# Autodesk Inventor assembly: iceTubeClockAssembly
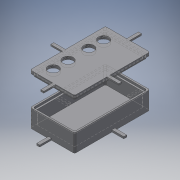
[picture p0: Inventor's stored thumbnail of the model, 180x180]
Saved by Autodesk Inventor 2016 (Build 200138000, 138)
## iProperties
Created: 2016-04-01
Part Number: iceTubeClockAssembly
Document SubType Name: Assembly
Designer: boztalay
Author: boztalay
## Documents named in this file (3)
- \\engin-labs.m.storage.umich.edu\boztalay\iceTubeClockAssembly.iam
- \\engin-labs.m.storage.umich.edu\boztalay\iceTubeClockBase.ipt
- \\engin-labs.m.storage.umich.edu\boztalay\iceTubeClockTop.ipt
## Components (2 placed, 2 different names)
1. iceTubeClockBase:1 — Mate:1, Flush:1, Flush:2
2. iceTubeClockTop:1 — Mate:1, Flush:1, Flush:2
## Relationships (3: Flush 2, Mate 1)
- Mate:1 (63.5 mm): iceTubeClockBase:1 ↔ iceTubeClockTop:1
- Flush:1: iceTubeClockBase:1 ↔ iceTubeClockTop:1
- Flush:2: iceTubeClockBase:1 ↔ iceTubeClockTop:1
